# Autodesk Inventor assembly: LinearDriveExample
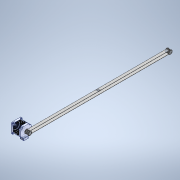
[picture p0: Inventor's stored thumbnail of the model, 180x180]
Saved by Autodesk Inventor 2022 (Build 260153000, 153)
## iProperties
Created: 2021-07-06
Part Number: LinearDriveExample
Document SubType Name: Assembly
Designer: jamieson-bl
Author: jamieson-bl
## Documents named in this file (4)
- \\Mac\Home\Desktop\WinnipegPMTTestFacility\LinearDriveExample.iam
- \\Mac\Home\Desktop\WinnipegPMTTestFacility\GPA20MR3150-A-HUC_Autodesk_Inventor_2020_20210706\AIS2020\GPA20MR3150-A-HUC.iam
- \\Mac\Home\Desktop\WinnipegPMTTestFacility\PKP266.ipt
- \\Mac\Home\Desktop\WinnipegPMTTestFacility\GBN1587MR3-150_Autodesk_Inventor_2020_20210706\GBN1587MR3-150_info-1-16-16.ipt
## Components (4 placed, 3 different names)
1. GPA20MR3150-A-HUC:1 [sub-assembly] — Mate:2, Flush:1, Mate:3, Mate:4
2. GPA20MR3150-A-HUC:2 [sub-assembly] — Flush:1, Mate:5
3. PKP266:1 — Mate:2
4. GBN1587MR3-150_info-1-16-16:1 — Mate:3, Mate:4, Mate:5
## Relationships (5: Mate 4, Flush 1)
- Mate:2: GPA20MR3150-A-HUC:1 ↔ PKP266:1
- Flush:1: GPA20MR3150-A-HUC:1 ↔ GPA20MR3150-A-HUC:2
- Mate:3: GPA20MR3150-A-HUC:1 ↔ GBN1587MR3-150_info-1-16-16:1
- Mate:4: GPA20MR3150-A-HUC:1 ↔ GBN1587MR3-150_info-1-16-16:1
- Mate:5: GPA20MR3150-A-HUC:2 ↔ GBN1587MR3-150_info-1-16-16:1
